# Autodesk Inventor assembly: quadcopter
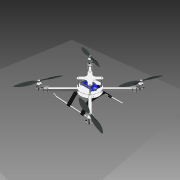
[picture p0: Inventor's stored thumbnail of the model, 180x180]
Saved by Autodesk Inventor 2013 (Build 170138000, 138)
## iProperties
Created: 2011-07-18
Part Number: quadcopter
Document SubType Name: Assembly
Designer: Nathan
Author: Nathan
## Documents named in this file (21)
- C:\Users\Nathan\Desktop\Dropbox\Quadcopter\quadcopter.iam
- C:\Users\Nathan\Desktop\Dropbox\Quadcopter\Arm.ipt
- C:\Users\Nathan\Desktop\Dropbox\Quadcopter\BaseTop.ipt
- C:\Users\Nathan\Desktop\Dropbox\Quadcopter\BaseBottom.ipt
- C:\Users\Nathan\Desktop\Dropbox\Quadcopter\MotorMount.iam
- C:\Users\Nathan\Documents\Inventor\Quadcopter\standoffiPart.ipt
- C:\Users\Nathan\Documents\Inventor\Quadcopter_Synced (USE ME IDIOT)\Quadcopter\standoffs\standoffiPart-021.ipt
- C:\Users\Nathan\Documents\Inventor\Content Center Files\R2011\en-US\ANSI B18.6.3(26)\ANSI B18.6.3 - 8-32 UNC - 1.25(7).ipt
- C:\Users\Nathan\Documents\Inventor\Content Center Files\R2011\en-US\ANSI B18.6.3(26)\ANSI B18.6.3 - 8-32 UNC - 1.125(7).ipt
- C:\Users\Nathan\Desktop\Dropbox\Quadcopter\LandingGear.iam
- C:\Users\Nathan\Desktop\Dropbox\Quadcopter\TopPlate.ipt
- C:\Users\Nathan\Documents\Inventor\Content Center Files\R2011\en-US\ANSI B18.6.3(26)\ANSI B18.6.3 - 8-32 UNC - 0.5(7).ipt
- C:\Users\Nathan\Documents\Inventor\Content Center Files\R2011\en-US\ANSI B18.6.3(26)\ANSI B18.6.3 - 4-40 UNC - 0.625(7).ipt
- C:\Users\Nathan\Desktop\Dropbox\Quadcopter\Motor.iam
- C:\Users\Nathan\Desktop\Dropbox\Quadcopter\propeller.iam
- C:\Users\Nathan\Documents\Inventor\Content Center Files\R2011\en-US\ANSI B18.6.3(26)\ANSI B18.6.3 - 6-32 UNC - 0.5625(7).ipt
- C:\Users\Nathan\Documents\Inventor\Content Center Files\R2011\en-US\ANSI B18.6.3(26)\ANSI B18.6.3 - 8-32 UNC - 1.375(7).ipt
- C:\Users\Nathan\Documents\Inventor\Content Center Files\R2011\en-US\ANSI B18.6.3(26)\ANSI B18.6.3 - 6-32 UNC - 0.5(7).ipt
- C:\Users\Nathan\Desktop\Dropbox\Quadcopter\Spacer_8-32.ipt
- C:\Users\Nathan\Desktop\Dropbox\Quadcopter\Spacer_4-40.ipt
- C:\Users\Nathan\Desktop\Dropbox\Quadcopter\arduinoWithShield.iam
## Components (57 placed, 19 different names)
1. BaseTop:1 — Mate:3, Mate:4, Mate:13, Mate:14, Mate:16, Mate:18, Mate:24, Mate:25, Mate:46, Mate:47, Mate:48, Mate:49, Mate:55, Mate:57, Mate:59, Mate:61, Mate:109, Mate:110, Mate:111, Mate:112, Mate:171, Mate:176, Mate:177, Mate:178, Mate:179, Angle:2, Mate:181, Angle:6, Angle:7
2. BaseBottom:1 — Mate:13, Mate:14, Mate:17, Mate:19, Mate:26, Mate:27, Mate:50, Mate:51, Mate:52, Mate:53, Mate:63, Mate:113, Mate:114, Mate:115, Mate:148, Mate:149, Mate:150, Mate:151, Mate:152, Mate:153, Mate:154, Mate:155, Mate:171
3. Cross Recessed Pan Head Machine Screw - Type II - Inch No. 8 - 32 - 1 1/4:1 — Mate:16, Mate:17, Mate:54
4. Cross Recessed Pan Head Machine Screw - Type II - Inch No. 8 - 32 - 1 1/8:2 — Mate:18, Mate:19
5. Cross Recessed Pan Head Machine Screw - Type II - Inch No. 8 - 32 - 1 1/4:7 — Mate:24, Mate:26, Mate:56, Mate:166
6. Cross Recessed Pan Head Machine Screw - Type II - Inch No. 8 - 32 - 1 1/8:3 — Mate:25, Mate:27, Mate:163
7. Cross Recessed Pan Head Machine Screw - Type II - Inch No. 8 - 32 - 1 3/8:1 — Mate:46, Mate:51, Mate:58
8. Cross Recessed Pan Head Machine Screw - Type II - Inch No. 8 - 32 - 1 1/8:4 — Mate:48, Mate:52
9. Cross Recessed Pan Head Machine Screw - Type II - Inch No. 8 - 32 - 1 1/4:2 — Mate:49, Mate:53, Mate:60
10. Cross Recessed Pan Head Machine Screw - Type II - Inch No. 8 - 32 - 1 1/8:1 — Mate:47, Mate:50
11. standoffiPart-021:5 — Mate:58, Mate:59, Mate:117, Mate:118
12. standoffiPart-021:6 — Mate:54, Mate:55
13. standoffiPart-021:7 — Mate:56, Mate:57
14. standoffiPart-021:8 — Mate:60, Mate:61, Mate:116
15. Cross Recessed Pan Head Machine Screw - Type II - Inch No. 4 - 40 - 5/8:2 — Mate:109, Mate:175
16. Cross Recessed Pan Head Machine Screw - Type II - Inch No. 4 - 40 - 5/8:4 — Mate:112, Mate:174
17. Cross Recessed Pan Head Machine Screw - Type II - Inch No. 4 - 40 - 5/8:1 — Mate:111, Mate:172
18. Cross Recessed Pan Head Machine Screw - Type II - Inch No. 4 - 40 - 5/8:3 — Mate:110, Mate:173
19. LandingGear:1 [sub-assembly] — Mate:113, Mate:114, Mate:115
20. TopPlate:1 — Mate:116, Mate:117, Mate:118, Mate:119, Mate:120, Mate:121, Mate:122, Mate:123, Mate:124, Mate:125, Mate:126, Mate:181
21. Cross Recessed Pan Head Machine Screw - Type II - Inch No. 8 - 32 - 1/2:1 — Mate:119, Mate:126
22. Cross Recessed Pan Head Machine Screw - Type II - Inch No. 8 - 32 - 1/2:2 — Mate:120, Mate:123
23. Cross Recessed Pan Head Machine Screw - Type II - Inch No. 8 - 32 - 1/2:3 — Mate:122, Mate:124
24. Cross Recessed Pan Head Machine Screw - Type II - Inch No. 8 - 32 - 1/2:4 — Mate:121, Mate:125
25. Cross Recessed Pan Head Machine Screw - Type II - Inch No. 6 - 32 - 1/2:1 — Mate:148, Mate:149
26. Cross Recessed Pan Head Machine Screw - Type II - Inch No. 6 - 32 - 9/16:4 — Mate:154, Mate:155
27. Cross Recessed Pan Head Machine Screw - Type II - Inch No. 6 - 32 - 9/16:3 — Mate:152, Mate:153
28. Cross Recessed Pan Head Machine Screw - Type II - Inch No. 6 - 32 - 9/16:1 — Mate:150, Mate:151
29. Spacer_4-40:1 — Mate:173, Mate:179
30. Spacer_4-40:2 — Mate:172, Mate:178, Mate:182, Mate:183
31. Spacer_4-40:3 — Mate:175, Mate:177
32. Spacer_4-40:4 — Mate:174, Mate:176
33. arduinoWithShield:1 [sub-assembly] — Mate:182, Mate:183, Angle:8
34. Arm:3 — Mate:3, Mate:4, Flush:22, Mate:22, Flush:24, Mate:63, Mate:164, Mate:165, Angle:2
35. Motor:3 [sub-assembly] — Mate:142, Mate:143, Mate:144
36. MotorMount:3 [sub-assembly] — Flush:22, Mate:22, Flush:24, Mate:142, Mate:143
37. propeller:1 [sub-assembly] — Mate:144
38. Spacer_8-32:3 — Mate:163, Mate:164
39. Spacer_8-32:4 — Mate:165, Mate:166
40. Arm:4
41. Motor:4 [sub-assembly]
42. MotorMount:4 [sub-assembly]
43. propeller:2 [sub-assembly]
44. Spacer_8-32:5
45. Spacer_8-32:8
46. Arm:5
47. Motor:5 [sub-assembly]
48. MotorMount:5 [sub-assembly]
49. propeller:3 [sub-assembly]
50. Spacer_8-32:6
51. Spacer_8-32:9
52. Arm:6
53. Motor:6 [sub-assembly]
54. MotorMount:6 [sub-assembly]
55. propeller:4 [sub-assembly]
56. Spacer_8-32:7
57. Spacer_8-32:10
## Component patterns: (4 elements, first: Arm:3 + Motor:3 + MotorMount:3 + propeller:1 + Spacer_8-32:3 + Spacer_8-32:4)
## Relationships (81: Mate 75, Angle 4, Flush 2)
- Mate:3: BaseTop:1 ↔ Arm:3
- Mate:4: BaseTop:1 ↔ Arm:3
- Mate:13: BaseTop:1 ↔ BaseBottom:1
- Mate:14: BaseTop:1 ↔ BaseBottom:1
- Mate:16: BaseTop:1 ↔ Cross Recessed Pan Head Machine Screw - Type II - Inch No. 8 - 32 - 1 1/4:1
- Mate:17: BaseBottom:1 ↔ Cross Recessed Pan Head Machine Screw - Type II - Inch No. 8 - 32 - 1 1/4:1
- Mate:18: BaseTop:1 ↔ Cross Recessed Pan Head Machine Screw - Type II - Inch No. 8 - 32 - 1 1/8:2
- Mate:19: BaseBottom:1 ↔ Cross Recessed Pan Head Machine Screw - Type II - Inch No. 8 - 32 - 1 1/8:2
- Flush:22: Arm:3 ↔ MotorMount:3
- Mate:22: Arm:3 ↔ MotorMount:3
- Mate:24: BaseTop:1 ↔ Cross Recessed Pan Head Machine Screw - Type II - Inch No. 8 - 32 - 1 1/4:7
- Mate:25: BaseTop:1 ↔ Cross Recessed Pan Head Machine Screw - Type II - Inch No. 8 - 32 - 1 1/8:3
- Mate:26: BaseBottom:1 ↔ Cross Recessed Pan Head Machine Screw - Type II - Inch No. 8 - 32 - 1 1/4:7
- Mate:27: BaseBottom:1 ↔ Cross Recessed Pan Head Machine Screw - Type II - Inch No. 8 - 32 - 1 1/8:3
- Flush:24: Arm:3 ↔ MotorMount:3
- Mate:46: BaseTop:1 ↔ Cross Recessed Pan Head Machine Screw - Type II - Inch No. 8 - 32 - 1 3/8:1
- Mate:47: BaseTop:1 ↔ Cross Recessed Pan Head Machine Screw - Type II - Inch No. 8 - 32 - 1 1/8:1
- Mate:48: BaseTop:1 ↔ Cross Recessed Pan Head Machine Screw - Type II - Inch No. 8 - 32 - 1 1/8:4
- Mate:49: BaseTop:1 ↔ Cross Recessed Pan Head Machine Screw - Type II - Inch No. 8 - 32 - 1 1/4:2
- Mate:50: BaseBottom:1 ↔ Cross Recessed Pan Head Machine Screw - Type II - Inch No. 8 - 32 - 1 1/8:1
- Mate:51: BaseBottom:1 ↔ Cross Recessed Pan Head Machine Screw - Type II - Inch No. 8 - 32 - 1 3/8:1
- Mate:52: BaseBottom:1 ↔ Cross Recessed Pan Head Machine Screw - Type II - Inch No. 8 - 32 - 1 1/8:4
- Mate:53: BaseBottom:1 ↔ Cross Recessed Pan Head Machine Screw - Type II - Inch No. 8 - 32 - 1 1/4:2
- Mate:54: Cross Recessed Pan Head Machine Screw - Type II - Inch No. 8 - 32 - 1 1/4:1 ↔ standoffiPart-021:6
- Mate:55: BaseTop:1 ↔ standoffiPart-021:6
- Mate:56: Cross Recessed Pan Head Machine Screw - Type II - Inch No. 8 - 32 - 1 1/4:7 ↔ standoffiPart-021:7
- Mate:57: BaseTop:1 ↔ standoffiPart-021:7
- Mate:58: Cross Recessed Pan Head Machine Screw - Type II - Inch No. 8 - 32 - 1 3/8:1 ↔ standoffiPart-021:5
- Mate:59: BaseTop:1 ↔ standoffiPart-021:5
- Mate:60: Cross Recessed Pan Head Machine Screw - Type II - Inch No. 8 - 32 - 1 1/4:2 ↔ standoffiPart-021:8
- Mate:61: BaseTop:1 ↔ standoffiPart-021:8
- Mate:63: BaseBottom:1 ↔ Arm:3
- Mate:109: BaseTop:1 ↔ Cross Recessed Pan Head Machine Screw - Type II - Inch No. 4 - 40 - 5/8:2
- Mate:110: BaseTop:1 ↔ Cross Recessed Pan Head Machine Screw - Type II - Inch No. 4 - 40 - 5/8:3
- Mate:111: BaseTop:1 ↔ Cross Recessed Pan Head Machine Screw - Type II - Inch No. 4 - 40 - 5/8:1
- Mate:112: BaseTop:1 ↔ Cross Recessed Pan Head Machine Screw - Type II - Inch No. 4 - 40 - 5/8:4
- Mate:113: BaseBottom:1 ↔ LandingGear:1
- Mate:114: BaseBottom:1 ↔ LandingGear:1
- Mate:115 (3.175 mm): BaseBottom:1 ↔ LandingGear:1
- Mate:116: standoffiPart-021:8 ↔ TopPlate:1
- Mate:117: standoffiPart-021:5 ↔ TopPlate:1
- Mate:118: standoffiPart-021:5 ↔ TopPlate:1
- Mate:119: TopPlate:1 ↔ Cross Recessed Pan Head Machine Screw - Type II - Inch No. 8 - 32 - 1/2:1
- Mate:120: TopPlate:1 ↔ Cross Recessed Pan Head Machine Screw - Type II - Inch No. 8 - 32 - 1/2:2
- Mate:121: TopPlate:1 ↔ Cross Recessed Pan Head Machine Screw - Type II - Inch No. 8 - 32 - 1/2:4
- Mate:122: TopPlate:1 ↔ Cross Recessed Pan Head Machine Screw - Type II - Inch No. 8 - 32 - 1/2:3
- Mate:123: TopPlate:1 ↔ Cross Recessed Pan Head Machine Screw - Type II - Inch No. 8 - 32 - 1/2:2
- Mate:124: TopPlate:1 ↔ Cross Recessed Pan Head Machine Screw - Type II - Inch No. 8 - 32 - 1/2:3
- Mate:125: TopPlate:1 ↔ Cross Recessed Pan Head Machine Screw - Type II - Inch No. 8 - 32 - 1/2:4
- Mate:126: TopPlate:1 ↔ Cross Recessed Pan Head Machine Screw - Type II - Inch No. 8 - 32 - 1/2:1
- Mate:142: Motor:3 ↔ MotorMount:3
- Mate:143: Motor:3 ↔ MotorMount:3
- Mate:144: Motor:3 ↔ propeller:1
- Mate:148: BaseBottom:1 ↔ Cross Recessed Pan Head Machine Screw - Type II - Inch No. 6 - 32 - 1/2:1
- Mate:149: BaseBottom:1 ↔ Cross Recessed Pan Head Machine Screw - Type II - Inch No. 6 - 32 - 1/2:1
- Mate:150: BaseBottom:1 ↔ Cross Recessed Pan Head Machine Screw - Type II - Inch No. 6 - 32 - 9/16:1
- Mate:151: BaseBottom:1 ↔ Cross Recessed Pan Head Machine Screw - Type II - Inch No. 6 - 32 - 9/16:1
- Mate:152: BaseBottom:1 ↔ Cross Recessed Pan Head Machine Screw - Type II - Inch No. 6 - 32 - 9/16:3
- Mate:153: BaseBottom:1 ↔ Cross Recessed Pan Head Machine Screw - Type II - Inch No. 6 - 32 - 9/16:3
- Mate:154: BaseBottom:1 ↔ Cross Recessed Pan Head Machine Screw - Type II - Inch No. 6 - 32 - 9/16:4
- Mate:155: BaseBottom:1 ↔ Cross Recessed Pan Head Machine Screw - Type II - Inch No. 6 - 32 - 9/16:4
- Mate:163: Cross Recessed Pan Head Machine Screw - Type II - Inch No. 8 - 32 - 1 1/8:3 ↔ Spacer_8-32:3
- Mate:164: Arm:3 ↔ Spacer_8-32:3
- Mate:165: Arm:3 ↔ Spacer_8-32:4
- Mate:166: Cross Recessed Pan Head Machine Screw - Type II - Inch No. 8 - 32 - 1 1/4:7 ↔ Spacer_8-32:4
- Mate:171 (22.225 mm): BaseTop:1 ↔ BaseBottom:1
- Mate:172: Cross Recessed Pan Head Machine Screw - Type II - Inch No. 4 - 40 - 5/8:1 ↔ Spacer_4-40:2
- Mate:173: Cross Recessed Pan Head Machine Screw - Type II - Inch No. 4 - 40 - 5/8:3 ↔ Spacer_4-40:1
- Mate:174: Cross Recessed Pan Head Machine Screw - Type II - Inch No. 4 - 40 - 5/8:4 ↔ Spacer_4-40:4
- Mate:175: Cross Recessed Pan Head Machine Screw - Type II - Inch No. 4 - 40 - 5/8:2 ↔ Spacer_4-40:3
- Mate:176: BaseTop:1 ↔ Spacer_4-40:4
- Mate:177: BaseTop:1 ↔ Spacer_4-40:3
- Mate:178: BaseTop:1 ↔ Spacer_4-40:2
- Mate:179: BaseTop:1 ↔ Spacer_4-40:1
- Angle:2 (180 deg): BaseTop:1 ↔ Arm:3
- Mate:181 (50.8 mm): BaseTop:1 ↔ TopPlate:1
- Angle:6 (0 deg): BaseTop:1
- Angle:7 (0 deg): BaseTop:1
- Mate:182: Spacer_4-40:2 ↔ arduinoWithShield:1
- Mate:183: Spacer_4-40:2 ↔ arduinoWithShield:1
- Angle:8 (-180 deg): arduinoWithShield:1
